# Autodesk Inventor assembly: Tape Measure Bracket Assembly V3
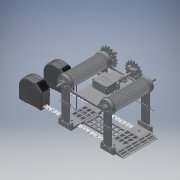
[picture p0: Inventor's stored thumbnail of the model, 180x180]
Saved by Autodesk Inventor 2019 (Build 230136000, 136)
## iProperties
Created: 2018-11-08
Part Number: Tape Measure Bracket Assembly V3
Document SubType Name: Assembly
Designer: Ashley
Author: Ashley
## Documents named in this file (20)
- C:\Users\Ashley\Desktop\repositories\design\inventor\2018-2019\Tape Measure Braket\Version Three\Tape Measure Bracket Assembly V3.iam
- C:\Users\Ashley\Desktop\repositories\design\inventor\2018-2019\Tape Measure Braket\Version Three\Bracket Bottom V3.ipt
- C:\Users\Ashley\Desktop\repositories\design\inventor\2018-2019\Tape Measure Braket\Tape Measure\Tape Measure Edited.iam
- C:\Users\Ashley\Desktop\repositories\design\inventor\2018-2019\Tape Measure Braket\Version Three\Side V3.ipt
- C:\Users\Ashley\Desktop\repositories\design\inventor\Imported Components\goBilda\Bearing6mmID.ipt
- C:\Users\Ashley\Desktop\repositories\design\inventor\2018-2019\Tape Measure Braket\Version Three\Pulley Left V3.ipt
- C:\Users\Ashley\Desktop\repositories\design\inventor\Imported Components\goBilda\DShaft140mm.ipt
- C:\Users\Ashley\Desktop\repositories\design\inventor\Imported Components\goBilda\Collar6mm\SetScrewCollar6mmboreassembly.iam
- C:\Users\Ashley\Desktop\repositories\design\inventor\Imported Components\goBilda\DShaft160mm.ipt
- C:\Users\Ashley\Desktop\repositories\design\inventor\2018-2019\Tape Measure Braket\Finished Parts\2mmAxel.ipt
- C:\Users\Ashley\Desktop\repositories\design\inventor\Imported Components\goBilda\CampingHub\ClampingHub assembly.iam
- C:\Users\Ashley\Desktop\repositories\design\inventor\Imported Components\goBilda\8mmPlasticPitchSproket.ipt
- C:\Users\Ashley\Desktop\repositories\design\inventor\Imported Components\goBilda\Servo To Shaft\ServoToShaftCoupler.iam
- C:\Users\Ashley\Desktop\repositories\design\inventor\2018-2019\Tape Measure Braket\Version Three\Braket Top V3.ipt
- C:\Users\Ashley\Desktop\repositories\design\inventor\2018-2019\Tape Measure Braket\Finished Parts\2mmAxel3in.ipt
- C:\Users\Ashley\Desktop\repositories\design\inventor\2018-2019\Tape Measure Braket\Version Three\Pulley Right V3.ipt
- C:\Users\Ashley\Desktop\repositories\design\inventor\Imported Components\REV\Motors and Servos\Rev_Servo.iam
- C:\Users\Ashley\Desktop\repositories\design\inventor\2018-2019\Tape Measure Braket\Version Three\Servo Plate V3.ipt
- C:\Users\Ashley\Desktop\repositories\design\inventor\2018-2019\Tape Measure Braket\Version Three\Servo Locks V3.ipt
- C:\Users\Ashley\Desktop\repositories\design\inventor\Imported Components\goBilda\DShaft40mm.ipt
## Components (38 placed, 32 different names)
1. Bracket Bottom — Mate:1, Mate:4, Mate:5, Insert:24, Mate:7
2. Tape Measure Right [sub-assembly]
3. Tape Measure Left [sub-assembly]
4. Back Right Side
5. Front Right Side — Mate:1, Insert:2, Insert:11
6. Front Left Side — Insert:3, Insert:10, Mate:8
7. Back Right Bearing — Insert:17
8. Front Right Bearing — Insert:2
9. Front Left Beaing — Insert:3
10. Front Left BEaring
11. Front Right Collar [sub-assembly]
12. Front Axel — Insert:8, Insert:25
13. Front Left Collar [sub-assembly] — Insert:8
14. Back Left Collar [sub-assembly]
15. Back Right Collar [sub-assembly] — Insert:18
16. Back Axel — Insert:17, Insert:18, Insert:19, Insert:26
17. Left axel — Insert:10
18. Right Axel — Insert:11
19. Back Sproket
20. Back Clamping Hub [sub-assembly] — Insert:19
21. Braket Top V3:1 — Mate:5
22. Braket Top V3:2 — Mate:4
23. Braket Top V3:3
24. Braket Top V3:4
25. 2mmAxel3in:1 — Insert:24
26. Pulley Right V3:1 — Insert:25, Mate:6
27. Pulley Right V3:2 — Insert:26, Symmetry:1
28. Pulley Left V3:1 — Mate:6
29. Pulley Left V3:2 — Symmetry:1
30. Side V3:4 — Mate:7
31. Servo Locks V3:1 — Mate:9
32. Servo Locks V3:2 — Mate:10, Mate:11
33. Servo Plate V3:1 — Mate:8, Mate:9, Mate:10
34. Rev_Servo:1 [sub-assembly] — Mate:11, Insert:27
35. ServoToShaftCoupler:1 [sub-assembly] — Insert:27, Insert:28
36. DShaft40mm:1 — Insert:28, Insert:30
37. 8mmPlasticPitchSproket:3 — Insert:29
38. ClampingHub assembly:3 [sub-assembly] — Insert:29, Insert:30
## Relationships (26: Insert 16, Mate 9, Symmetry 1)
- Mate:1: Bracket Bottom ↔ Front Right Side
- Insert:2: Front Right Side ↔ Front Right Bearing
- Insert:3: Front Left Side ↔ Front Left Beaing
- Insert:8 (14 mm): Front Axel ↔ Front Left Collar
- Insert:10 (-30 mm): Front Left Side ↔ Left axel
- Insert:11 (-30 mm): Front Right Side ↔ Right Axel
- [Insert] (-1 mm): Back Sproket ↔ Back Clamping Hub
- Insert:17 (20 mm): Back Right Bearing ↔ Back Axel
- Insert:18 (12 mm): Back Right Collar ↔ Back Axel
- Insert:19 (11 mm): Back Axel ↔ Back Clamping Hub
- Mate:4: Bracket Bottom ↔ Braket Top V3:2
- Mate:5: Bracket Bottom ↔ Braket Top V3:1
- Insert:24 (-6.5 mm): Bracket Bottom ↔ 2mmAxel3in:1
- Insert:25 (30 mm): Front Axel ↔ Pulley Right V3:1
- Mate:6: Pulley Right V3:1 ↔ Pulley Left V3:1
- Insert:26 (39 mm): Back Axel ↔ Pulley Right V3:2
- Symmetry:1: Pulley Right V3:2 ↔ Pulley Left V3:2
- Mate:7: Bracket Bottom ↔ Side V3:4
- Mate:8: Front Left Side ↔ Servo Plate V3:1
- Mate:9: Servo Locks V3:1 ↔ Servo Plate V3:1
- Mate:10: Servo Locks V3:2 ↔ Servo Plate V3:1
- Mate:11: Servo Locks V3:2 ↔ Rev_Servo:1
- Insert:27 (0.4 mm): Rev_Servo:1 ↔ ServoToShaftCoupler:1
- Insert:28 (-10 mm): ServoToShaftCoupler:1 ↔ DShaft40mm:1
- Insert:29 (-1 mm): 8mmPlasticPitchSproket:3 ↔ ClampingHub assembly:3
- Insert:30 (-11 mm): DShaft40mm:1 ↔ ClampingHub assembly:3
## Named parameters: d26_d25 = -1 mm
